# Autodesk Inventor assembly: Mock Module PCB - v1p4b
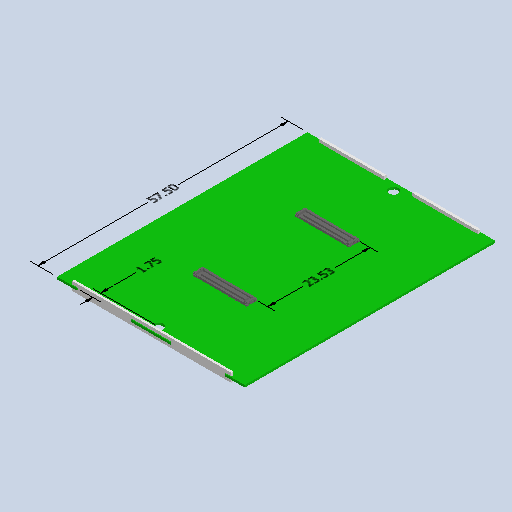
[picture p0: Inventor's stored thumbnail of the model, 512x512]
Saved by Autodesk Inventor 2023 (Build 270158000, 158)
## iProperties
Created: 2021-07-19
Part Number: Mock Module PCB - v1p4b
Document SubType Name: Assembly
Designer: Caleb
Author: Caleb
## Documents named in this file (5)
- C:\Users\Caleb\Desktop\nebraska-silicon-lab\Hardware\ETL\modules\tamale v1.4\Mock Module PCB - v1p4b.iam
- C:\Users\Caleb\Desktop\nebraska-silicon-lab\Hardware\ETL\ETL-SH-Design\3D-model\K3D-WP7B-S050VA1-V3_JAE_Proprietary v1_14.iam
- C:\Users\Caleb\Desktop\nebraska-silicon-lab\Hardware\ETL\modules\tamale v1.4\Mock Module PCB - v1p4.ipt
- C:\Users\Caleb\Desktop\nebraska-silicon-lab\Hardware\ETL\modules\tamale v1.4\insert spacer - v1.ipt
- C:\Users\Caleb\Desktop\nebraska-silicon-lab\Hardware\ETL\modules\tamale v1.4\insert spacer - v2.ipt
## Components (6 placed, 4 different names)
1. Mock Module PCB - v1p4:1 — Mate:1, Mate:2, Flush:4, Flush:6, Mate:10, Mate:11, Mate:12, Mate:13, Mate:14, Mate:15, Mate:16, Mate:17, Mate:18
2. K3D-WP7B-S050VA1-V3_JAE_Proprietary v1_14:1 [sub-assembly] — Mate:1, Flush:3, Flush:5
3. K3D-WP7B-S050VA1-V3_JAE_Proprietary v1_14:2 [sub-assembly] — Mate:2, Flush:3, Flush:4, Flush:5, Flush:6
4. insert spacer - v1:3 — Mate:10, Mate:13, Mate:14
5. insert spacer - v1:4 — Mate:11, Mate:12, Mate:15
6. insert spacer - v2:1 — Mate:16, Mate:17, Mate:18
## Relationships (15: Mate 11, Flush 4)
- Mate:1: Mock Module PCB - v1p4:1 ↔ K3D-WP7B-S050VA1-V3_JAE_Proprietary v1_14:1
- Mate:2: Mock Module PCB - v1p4:1 ↔ K3D-WP7B-S050VA1-V3_JAE_Proprietary v1_14:2
- Flush:3 (23.531 mm): K3D-WP7B-S050VA1-V3_JAE_Proprietary v1_14:1 ↔ K3D-WP7B-S050VA1-V3_JAE_Proprietary v1_14:2
- Flush:4 (15.7945 mm): Mock Module PCB - v1p4:1 ↔ K3D-WP7B-S050VA1-V3_JAE_Proprietary v1_14:2
- Flush:5: K3D-WP7B-S050VA1-V3_JAE_Proprietary v1_14:1 ↔ K3D-WP7B-S050VA1-V3_JAE_Proprietary v1_14:2
- Flush:6 (15.307 mm): Mock Module PCB - v1p4:1 ↔ K3D-WP7B-S050VA1-V3_JAE_Proprietary v1_14:2
- Mate:10: Mock Module PCB - v1p4:1 ↔ insert spacer - v1:3
- Mate:11: Mock Module PCB - v1p4:1 ↔ insert spacer - v1:4
- Mate:12: Mock Module PCB - v1p4:1 ↔ insert spacer - v1:4
- Mate:13: Mock Module PCB - v1p4:1 ↔ insert spacer - v1:3
- Mate:14: Mock Module PCB - v1p4:1 ↔ insert spacer - v1:3
- Mate:15: Mock Module PCB - v1p4:1 ↔ insert spacer - v1:4
- Mate:16: Mock Module PCB - v1p4:1 ↔ insert spacer - v2:1
- Mate:17: Mock Module PCB - v1p4:1 ↔ insert spacer - v2:1
- Mate:18: Mock Module PCB - v1p4:1 ↔ insert spacer - v2:1
